# Autodesk Inventor assembly: Lower Frame
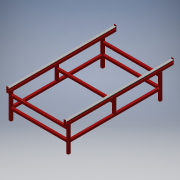
[picture p0: Inventor's stored thumbnail of the model, 180x180]
Saved by Autodesk Inventor 2018.2 (Build 222227000, 227)
## iProperties
Created: 2017-12-10
Part Number: Lower Frame
Document SubType Name: Assembly
Designer: torba
Author: torba
## Documents named in this file (13)
- C:\Users\torba\OneDrive\Documents\Inventor\Plasma 5x10\Lower Frame.iam
- C:\Users\torba\OneDrive\Documents\Inventor\Plasma 5x10\3 X 3 X .125 WALL SQ TUBE\3 X 3 X .125 WALL SQ TUBE-10.ipt
- C:\Users\torba\OneDrive\Documents\Inventor\Plasma 5x10\3 X 3 X .125 WALL SQ TUBE.ipt
- C:\Users\torba\OneDrive\Documents\Inventor\Plasma 5x10\3 X 3 X .125 WALL SQ TUBE\3 X 3 X .125 WALL SQ TUBE-02.ipt
- C:\Users\torba\OneDrive\Documents\Inventor\Plasma 5x10\3 X 3 X .125 WALL SQ TUBE\3 X 3 X .125 WALL SQ TUBE-06.ipt
- C:\Users\torba\OneDrive\Documents\Inventor\Plasma 5x10\3 X 3 X .125 WALL SQ TUBE\3 X 3 X .125 WALL SQ TUBE-13.ipt
- C:\Users\torba\OneDrive\Documents\Inventor\Plasma 5x10\3 X 3 X .125 WALL SQ TUBE\3 X 3 X .125 WALL SQ TUBE-12.ipt
- C:\Users\torba\OneDrive\Documents\Inventor\Plasma 5x10\0.25 X 3 HOT ROLLED STEEL.ipt
- C:\Users\torba\OneDrive\Documents\Inventor\Plasma 5x10\3-8 x 3 cold rolled steel\3-8 x 3 cold rolled steel-144.ipt
- C:\Users\torba\OneDrive\Documents\Inventor\Plasma 5x10\3-8 x 3 cold rolled steel.ipt
- C:\Users\torba\OneDrive\Documents\Inventor\Plasma 5x10\1.5 X 2 X .125 WALL SQ TUBE.ipt
- C:\Users\torba\OneDrive\Documents\Inventor\Plasma 5x10\RSHC10XX00 Rack (Simplified)\RSHC10XX00 Rack (Simplified)-130.ipt
- C:\Users\torba\OneDrive\Documents\Inventor\Plasma 5x10\RSHC10XX00 Rack (Simplified).ipt
## Components (25 placed, 9 different names)
1. 1.5 X 2 X .125 WALL SQ TUBE:2 — Mate:12, Flush:36, Flush:37, Mate:18
2. 1.5 X 2 X .125 WALL SQ TUBE:1 — Mate:11, Flush:35, Flush:38, Mate:19
3. 3 X 3 X .125 WALL SQ TUBE-12:1 — Mate:2, Flush:9, Flush:10, Flush:11, Flush:12, Mate:3, Flush:34, Mate:11, Flush:35, Flush:38, Mate:13, Mate:15, Mate:16, Flush:41, Flush:42, Flush:45, Flush:46
4. 3 X 3 X .125 WALL SQ TUBE-12:2 — Mate:1, Flush:6, Flush:7, Flush:8, Flush:12, Mate:4, Mate:12, Flush:36, Flush:37, Mate:14, Mate:17, Flush:39, Flush:40, Flush:43, Flush:44
5. 3 X 3 X .125 WALL SQ TUBE-02:3 — Flush:13, Flush:14, Flush:22, Flush:31, Flush:32, Flush:33, Mate:26
6. 3 X 3 X .125 WALL SQ TUBE-02:4 — Flush:13, Flush:20, Mate:3, Mate:4, Flush:32, Mate:13, Mate:26
7. 3 X 3 X .125 WALL SQ TUBE-06:5 — Mate:5, Flush:26, Mate:8, Flush:30, Mate:9
8. 3 X 3 X .125 WALL SQ TUBE-06:6 — Mate:6, Mate:7, Flush:25, Flush:28, Flush:29, Mate:10
9. 3 X 3 X .125 WALL SQ TUBE-02:7 — Flush:14, Flush:23, Flush:29, Flush:30
10. 3 X 3 X .125 WALL SQ TUBE-02:9 — Flush:17, Flush:24, Flush:33
11. 3 X 3 X .125 WALL SQ TUBE-02:10 — Flush:17, Flush:19, Flush:27, Flush:28, Mate:10
12. 3 X 3 X .125 WALL SQ TUBE-13:11 — Flush:3, Flush:10, Mate:5
13. 3 X 3 X .125 WALL SQ TUBE-13:12 — Flush:2, Flush:3, Flush:5, Mate:2, Flush:9, Flush:26, Mate:8, Flush:27, Flush:34
14. 3 X 3 X .125 WALL SQ TUBE-13:13 — Flush:1, Flush:2, Flush:7, Flush:23, Flush:24, Mate:6
15. 3 X 3 X .125 WALL SQ TUBE-13:14 — Flush:1, Mate:1, Flush:6, Flush:19, Flush:20, Mate:7, Flush:25
16. 3 X 3 X .125 WALL SQ TUBE-10:15 — Flush:4, Flush:5, Flush:11, Mate:9, Flush:31
17. 3 X 3 X .125 WALL SQ TUBE-10:16 — Flush:4, Flush:8, Flush:22
18. 0.25 X 3 HOT ROLLED STEEL:1 — Mate:14, Flush:43, Flush:44, Mate:21, Mate:27
19. 0.25 X 3 HOT ROLLED STEEL:2 — Mate:15, Flush:45, Flush:46, Mate:28
20. 0.25 X 3 HOT ROLLED STEEL:3 — Mate:16, Flush:41, Flush:42, Mate:20, Flush:47
21. 0.25 X 3 HOT ROLLED STEEL:4 — Mate:17, Flush:39, Flush:40, Flush:48
22. 3-8 x 3 cold rolled steel-144:1 — Mate:19, Mate:20, Flush:47, Mate:29, Flush:49
23. 3-8 x 3 cold rolled steel-144:2 — Mate:18, Flush:48, Mate:21, Mate:30, Flush:50
24. RSHC10XX00 Rack (Simplified)-130:1 — Mate:27, Mate:30, Flush:50
25. RSHC10XX00 Rack (Simplified)-130:2 — Mate:28, Mate:29, Flush:49
## Relationships (72: Flush 46, Mate 26)
- Flush:1: 3 X 3 X .125 WALL SQ TUBE-13:13 ↔ 3 X 3 X .125 WALL SQ TUBE-13:14
- Flush:2: 3 X 3 X .125 WALL SQ TUBE-13:12 ↔ 3 X 3 X .125 WALL SQ TUBE-13:13
- Flush:3: 3 X 3 X .125 WALL SQ TUBE-13:11 ↔ 3 X 3 X .125 WALL SQ TUBE-13:12
- Flush:4: 3 X 3 X .125 WALL SQ TUBE-10:15 ↔ 3 X 3 X .125 WALL SQ TUBE-10:16
- Flush:5: 3 X 3 X .125 WALL SQ TUBE-13:12 ↔ 3 X 3 X .125 WALL SQ TUBE-10:15
- Mate:1: 3 X 3 X .125 WALL SQ TUBE-12:2 ↔ 3 X 3 X .125 WALL SQ TUBE-13:14
- Flush:6: 3 X 3 X .125 WALL SQ TUBE-12:2 ↔ 3 X 3 X .125 WALL SQ TUBE-13:14
- Flush:7: 3 X 3 X .125 WALL SQ TUBE-12:2 ↔ 3 X 3 X .125 WALL SQ TUBE-13:13
- Flush:8: 3 X 3 X .125 WALL SQ TUBE-12:2 ↔ 3 X 3 X .125 WALL SQ TUBE-10:16
- Mate:2: 3 X 3 X .125 WALL SQ TUBE-12:1 ↔ 3 X 3 X .125 WALL SQ TUBE-13:12
- Flush:9: 3 X 3 X .125 WALL SQ TUBE-12:1 ↔ 3 X 3 X .125 WALL SQ TUBE-13:12
- Flush:10: 3 X 3 X .125 WALL SQ TUBE-12:1 ↔ 3 X 3 X .125 WALL SQ TUBE-13:11
- Flush:11: 3 X 3 X .125 WALL SQ TUBE-12:1 ↔ 3 X 3 X .125 WALL SQ TUBE-10:15
- Flush:12: 3 X 3 X .125 WALL SQ TUBE-12:1 ↔ 3 X 3 X .125 WALL SQ TUBE-12:2
- Flush:13: 3 X 3 X .125 WALL SQ TUBE-02:3 ↔ 3 X 3 X .125 WALL SQ TUBE-02:4
- Flush:14: 3 X 3 X .125 WALL SQ TUBE-02:3 ↔ 3 X 3 X .125 WALL SQ TUBE-02:7
- Flush:17: 3 X 3 X .125 WALL SQ TUBE-02:9 ↔ 3 X 3 X .125 WALL SQ TUBE-02:10
- Flush:19: 3 X 3 X .125 WALL SQ TUBE-02:10 ↔ 3 X 3 X .125 WALL SQ TUBE-13:14
- Flush:20: 3 X 3 X .125 WALL SQ TUBE-02:4 ↔ 3 X 3 X .125 WALL SQ TUBE-13:14
- Flush:22: 3 X 3 X .125 WALL SQ TUBE-02:3 ↔ 3 X 3 X .125 WALL SQ TUBE-10:16
- Flush:23: 3 X 3 X .125 WALL SQ TUBE-02:7 ↔ 3 X 3 X .125 WALL SQ TUBE-13:13
- Flush:24: 3 X 3 X .125 WALL SQ TUBE-02:9 ↔ 3 X 3 X .125 WALL SQ TUBE-13:13
- Mate:3: 3 X 3 X .125 WALL SQ TUBE-12:1 ↔ 3 X 3 X .125 WALL SQ TUBE-02:4
- Mate:4: 3 X 3 X .125 WALL SQ TUBE-12:2 ↔ 3 X 3 X .125 WALL SQ TUBE-02:4
- Mate:5: 3 X 3 X .125 WALL SQ TUBE-06:5 ↔ 3 X 3 X .125 WALL SQ TUBE-13:11
- Mate:6: 3 X 3 X .125 WALL SQ TUBE-06:6 ↔ 3 X 3 X .125 WALL SQ TUBE-13:13
- Mate:7: 3 X 3 X .125 WALL SQ TUBE-06:6 ↔ 3 X 3 X .125 WALL SQ TUBE-13:14
- Flush:25: 3 X 3 X .125 WALL SQ TUBE-06:6 ↔ 3 X 3 X .125 WALL SQ TUBE-13:14
- Flush:26: 3 X 3 X .125 WALL SQ TUBE-06:5 ↔ 3 X 3 X .125 WALL SQ TUBE-13:12
- Mate:8: 3 X 3 X .125 WALL SQ TUBE-06:5 ↔ 3 X 3 X .125 WALL SQ TUBE-13:12
- Flush:27: 3 X 3 X .125 WALL SQ TUBE-02:10 ↔ 3 X 3 X .125 WALL SQ TUBE-13:12
- Flush:28: 3 X 3 X .125 WALL SQ TUBE-06:6 ↔ 3 X 3 X .125 WALL SQ TUBE-02:10
- Flush:29: 3 X 3 X .125 WALL SQ TUBE-06:6 ↔ 3 X 3 X .125 WALL SQ TUBE-02:7
- Flush:30: 3 X 3 X .125 WALL SQ TUBE-06:5 ↔ 3 X 3 X .125 WALL SQ TUBE-02:7
- Mate:9: 3 X 3 X .125 WALL SQ TUBE-06:5 ↔ 3 X 3 X .125 WALL SQ TUBE-10:15
- Flush:31: 3 X 3 X .125 WALL SQ TUBE-02:3 ↔ 3 X 3 X .125 WALL SQ TUBE-10:15
- Flush:32: 3 X 3 X .125 WALL SQ TUBE-02:3 ↔ 3 X 3 X .125 WALL SQ TUBE-02:4
- Flush:33: 3 X 3 X .125 WALL SQ TUBE-02:3 ↔ 3 X 3 X .125 WALL SQ TUBE-02:9
- Flush:34 (76.2 mm): 3 X 3 X .125 WALL SQ TUBE-12:1 ↔ 3 X 3 X .125 WALL SQ TUBE-13:12
- Mate:10: 3 X 3 X .125 WALL SQ TUBE-06:6 ↔ 3 X 3 X .125 WALL SQ TUBE-02:10
- Mate:11: 1.5 X 2 X .125 WALL SQ TUBE:1 ↔ 3 X 3 X .125 WALL SQ TUBE-12:1
- Mate:12: 1.5 X 2 X .125 WALL SQ TUBE:2 ↔ 3 X 3 X .125 WALL SQ TUBE-12:2
- Flush:35: 1.5 X 2 X .125 WALL SQ TUBE:1 ↔ 3 X 3 X .125 WALL SQ TUBE-12:1
- Flush:36: 1.5 X 2 X .125 WALL SQ TUBE:2 ↔ 3 X 3 X .125 WALL SQ TUBE-12:2
- Flush:37 (19.05 mm): 1.5 X 2 X .125 WALL SQ TUBE:2 ↔ 3 X 3 X .125 WALL SQ TUBE-12:2
- Flush:38 (19.05 mm): 1.5 X 2 X .125 WALL SQ TUBE:1 ↔ 3 X 3 X .125 WALL SQ TUBE-12:1
- Mate:13 (76.2 mm): 3 X 3 X .125 WALL SQ TUBE-12:1 ↔ 3 X 3 X .125 WALL SQ TUBE-02:4
- Mate:14: 3 X 3 X .125 WALL SQ TUBE-12:2 ↔ 0.25 X 3 HOT ROLLED STEEL:1
- Mate:15: 3 X 3 X .125 WALL SQ TUBE-12:1 ↔ 0.25 X 3 HOT ROLLED STEEL:2
- Mate:16: 3 X 3 X .125 WALL SQ TUBE-12:1 ↔ 0.25 X 3 HOT ROLLED STEEL:3
- Mate:17: 3 X 3 X .125 WALL SQ TUBE-12:2 ↔ 0.25 X 3 HOT ROLLED STEEL:4
- Flush:39: 3 X 3 X .125 WALL SQ TUBE-12:2 ↔ 0.25 X 3 HOT ROLLED STEEL:4
- Flush:40: 3 X 3 X .125 WALL SQ TUBE-12:2 ↔ 0.25 X 3 HOT ROLLED STEEL:4
- Flush:41: 3 X 3 X .125 WALL SQ TUBE-12:1 ↔ 0.25 X 3 HOT ROLLED STEEL:3
- Flush:42: 3 X 3 X .125 WALL SQ TUBE-12:1 ↔ 0.25 X 3 HOT ROLLED STEEL:3
- Flush:43: 3 X 3 X .125 WALL SQ TUBE-12:2 ↔ 0.25 X 3 HOT ROLLED STEEL:1
- Flush:44: 3 X 3 X .125 WALL SQ TUBE-12:2 ↔ 0.25 X 3 HOT ROLLED STEEL:1
- Flush:45: 3 X 3 X .125 WALL SQ TUBE-12:1 ↔ 0.25 X 3 HOT ROLLED STEEL:2
- Flush:46: 3 X 3 X .125 WALL SQ TUBE-12:1 ↔ 0.25 X 3 HOT ROLLED STEEL:2
- Mate:18: 1.5 X 2 X .125 WALL SQ TUBE:2 ↔ 3-8 x 3 cold rolled steel-144:2
- Mate:19: 1.5 X 2 X .125 WALL SQ TUBE:1 ↔ 3-8 x 3 cold rolled steel-144:1
- Mate:20: 0.25 X 3 HOT ROLLED STEEL:3 ↔ 3-8 x 3 cold rolled steel-144:1
- Flush:47: 0.25 X 3 HOT ROLLED STEEL:3 ↔ 3-8 x 3 cold rolled steel-144:1
- Flush:48: 0.25 X 3 HOT ROLLED STEEL:4 ↔ 3-8 x 3 cold rolled steel-144:2
- Mate:21: 0.25 X 3 HOT ROLLED STEEL:1 ↔ 3-8 x 3 cold rolled steel-144:2
- Mate:26 (1485.9 mm): 3 X 3 X .125 WALL SQ TUBE-02:3 ↔ 3 X 3 X .125 WALL SQ TUBE-02:4
- Mate:27 (177.8 mm): 0.25 X 3 HOT ROLLED STEEL:1 ↔ RSHC10XX00 Rack (Simplified)-130:1
- Mate:28 (177.8 mm): 0.25 X 3 HOT ROLLED STEEL:2 ↔ RSHC10XX00 Rack (Simplified)-130:2
- Mate:29: 3-8 x 3 cold rolled steel-144:1 ↔ RSHC10XX00 Rack (Simplified)-130:2
- Flush:49: 3-8 x 3 cold rolled steel-144:1 ↔ RSHC10XX00 Rack (Simplified)-130:2
- Mate:30: 3-8 x 3 cold rolled steel-144:2 ↔ RSHC10XX00 Rack (Simplified)-130:1
- Flush:50: 3-8 x 3 cold rolled steel-144:2 ↔ RSHC10XX00 Rack (Simplified)-130:1
